(part 1 of 2)
# Autodesk Inventor assembly: ODrive S1 Housing Assembly
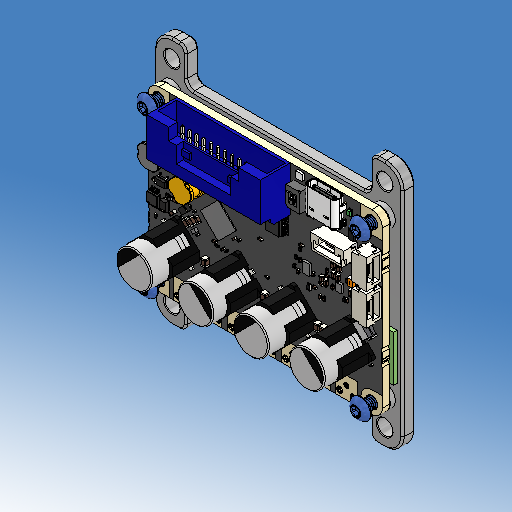
[picture p0: Inventor's stored thumbnail of the model, 512x512]
Saved by Autodesk Inventor 2025 (Build 290162000, 162)
## iProperties
Created: 2024-06-17
Part Number: ODrive S1 Housing Assembly
Description: STEP AP242
Document SubType Name: Assembly
Designer: seene
Title: 666fe0848788064f3eef2e7c
Preprocessor: ST-DEVELOPER v20
## Documents named in this file (550)
- C:\Users\seene\OneDrive\SBRT\Robocup Rescue\Chassis\Electronics Box\ODrive S1 Housing Assembly\ODrive S1 Housing Assembly.iam
- C:\Users\seene\OneDrive\SBRT\Robocup Rescue\Chassis\Electronics Box\ODrive S1 Housing Assembly\ODrive S1 Thermal Pad.ipt
- C:\Users\seene\OneDrive\SBRT\Robocup Rescue\Chassis\Electronics Box\ODrive S1 Housing Assembly\ODrive S1 Heatspreader.ipt
- C:\Users\seene\OneDrive\SBRT\Robocup Rescue\Chassis\Electronics Box\ODrive S1 Housing Assembly\90991A113_18-8 Stainless Steel Button Head Torx Screws.ipt
- C:\Users\seene\OneDrive\SBRT\Robocup Rescue\Chassis\Electronics Box\ODrive S1 Housing Assembly\ODrive S1 Cover.ipt
- C:\Users\seene\OneDrive\SBRT\Robocup Rescue\Chassis\Electronics Box\ODrive S1 Housing Assembly\C_0603_1608Metric_30.ipt
- C:\Users\seene\OneDrive\SBRT\Robocup Rescue\Chassis\Electronics Box\ODrive S1 Housing Assembly\C_0603_1608Metric_34.ipt
- C:\Users\seene\OneDrive\SBRT\Robocup Rescue\Chassis\Electronics Box\ODrive S1 Housing Assembly\C_0402_1005Metric_17.ipt
- C:\Users\seene\OneDrive\SBRT\Robocup Rescue\Chassis\Electronics Box\ODrive S1 Housing Assembly\C_0402_1005Metric_27.ipt
- C:\Users\seene\OneDrive\SBRT\Robocup Rescue\Chassis\Electronics Box\ODrive S1 Housing Assembly\C_0805_1MM_3.ipt
- C:\Users\seene\OneDrive\SBRT\Robocup Rescue\Chassis\Electronics Box\ODrive S1 Housing Assembly\_X2_8010632F54C130EA30FC30C97DDA03A6_X0_10_SIZE_CODE_G_4.ipt
- C:\Users\seene\OneDrive\SBRT\Robocup Rescue\Chassis\Electronics Box\ODrive S1 Housing Assembly\SOP_Advance(N)_(1)_7.ipt
- C:\Users\seene\OneDrive\SBRT\Robocup Rescue\Chassis\Electronics Box\ODrive S1 Housing Assembly\D_SOD-123F_3.ipt
- C:\Users\seene\OneDrive\SBRT\Robocup Rescue\Chassis\Electronics Box\ODrive S1 Housing Assembly\R_0402_1005Metric_63.ipt
- C:\Users\seene\OneDrive\SBRT\Robocup Rescue\Chassis\Electronics Box\ODrive S1 Housing Assembly\SOT23-3.ipt
- C:\Users\seene\OneDrive\SBRT\Robocup Rescue\Chassis\Electronics Box\ODrive S1 Housing Assembly\SOP_Advance(N)_(1)_2.ipt
- C:\Users\seene\OneDrive\SBRT\Robocup Rescue\Chassis\Electronics Box\ODrive S1 Housing Assembly\SOP_Advance(N)_(1)_5.ipt
- C:\Users\seene\OneDrive\SBRT\Robocup Rescue\Chassis\Electronics Box\ODrive S1 Housing Assembly\Open_CASCADE_STEP_translator_6.8_48.4.1_67.ipt
- C:\Users\seene\OneDrive\SBRT\Robocup Rescue\Chassis\Electronics Box\ODrive S1 Housing Assembly\R_0402_1005Metric_30.ipt
- C:\Users\seene\OneDrive\SBRT\Robocup Rescue\Chassis\Electronics Box\ODrive S1 Housing Assembly\R_0402_1005Metric_44.ipt
- C:\Users\seene\OneDrive\SBRT\Robocup Rescue\Chassis\Electronics Box\ODrive S1 Housing Assembly\R_0402_1005Metric_56.ipt
- C:\Users\seene\OneDrive\SBRT\Robocup Rescue\Chassis\Electronics Box\ODrive S1 Housing Assembly\Open_CASCADE_STEP_translator_6.8_48.4.1_3.ipt
- C:\Users\seene\OneDrive\SBRT\Robocup Rescue\Chassis\Electronics Box\ODrive S1 Housing Assembly\Open_CASCADE_STEP_translator_6.8_48.4.1_19.ipt
- C:\Users\seene\OneDrive\SBRT\Robocup Rescue\Chassis\Electronics Box\ODrive S1 Housing Assembly\Open_CASCADE_STEP_translator_6.8_48.4.1_35.ipt
- C:\Users\seene\OneDrive\SBRT\Robocup Rescue\Chassis\Electronics Box\ODrive S1 Housing Assembly\Open_CASCADE_STEP_translator_6.8_48.4.1_51.ipt
- C:\Users\seene\OneDrive\SBRT\Robocup Rescue\Chassis\Electronics Box\ODrive S1 Housing Assembly\LED_0603_APT1608_GREEN.ipt
- C:\Users\seene\OneDrive\SBRT\Robocup Rescue\Chassis\Electronics Box\ODrive S1 Housing Assembly\_X2_8010632F54C15EA7724803A6_X0_10_SIZE_CODE_G.ipt
- C:\Users\seene\OneDrive\SBRT\Robocup Rescue\Chassis\Electronics Box\ODrive S1 Housing Assembly\Open_CASCADE_STEP_translator_6.8_34.4.1_5.ipt
- C:\Users\seene\OneDrive\SBRT\Robocup Rescue\Chassis\Electronics Box\ODrive S1 Housing Assembly\Open_CASCADE_STEP_translator_6.8_41.4.1_2.ipt
- C:\Users\seene\OneDrive\SBRT\Robocup Rescue\Chassis\Electronics Box\ODrive S1 Housing Assembly\C_0402_1005Metric_8.ipt
- C:\Users\seene\OneDrive\SBRT\Robocup Rescue\Chassis\Electronics Box\ODrive S1 Housing Assembly\Cylinder_15.ipt
- C:\Users\seene\OneDrive\SBRT\Robocup Rescue\Chassis\Electronics Box\ODrive S1 Housing Assembly\SOT23-6.ipt
- C:\Users\seene\OneDrive\SBRT\Robocup Rescue\Chassis\Electronics Box\ODrive S1 Housing Assembly\C_0603_1608Metric_7.ipt
- C:\Users\seene\OneDrive\SBRT\Robocup Rescue\Chassis\Electronics Box\ODrive S1 Housing Assembly\Pins.ipt
- C:\Users\seene\OneDrive\SBRT\Robocup Rescue\Chassis\Electronics Box\ODrive S1 Housing Assembly\L_0603_1608Metric.ipt
- C:\Users\seene\OneDrive\SBRT\Robocup Rescue\Chassis\Electronics Box\ODrive S1 Housing Assembly\Open_CASCADE_STEP_translator_6.8_2.3.1_9.ipt
- C:\Users\seene\OneDrive\SBRT\Robocup Rescue\Chassis\Electronics Box\ODrive S1 Housing Assembly\Leader_2.ipt
- C:\Users\seene\OneDrive\SBRT\Robocup Rescue\Chassis\Electronics Box\ODrive S1 Housing Assembly\Open_CASCADE_STEP_translator_6.8_56.2.1.ipt
- C:\Users\seene\OneDrive\SBRT\Robocup Rescue\Chassis\Electronics Box\ODrive S1 Housing Assembly\Leader_4.ipt
- C:\Users\seene\OneDrive\SBRT\Robocup Rescue\Chassis\Electronics Box\ODrive S1 Housing Assembly\Leader_8.ipt
- C:\Users\seene\OneDrive\SBRT\Robocup Rescue\Chassis\Electronics Box\ODrive S1 Housing Assembly\C_0603_1608Metric_24.ipt
- C:\Users\seene\OneDrive\SBRT\Robocup Rescue\Chassis\Electronics Box\ODrive S1 Housing Assembly\D_SOD-123F.ipt
- C:\Users\seene\OneDrive\SBRT\Robocup Rescue\Chassis\Electronics Box\ODrive S1 Housing Assembly\_X2_8010632F54C15EA77248752888DC52A97AEF5B5003A6_X0_10_SIZE_CODE_G_3.ipt
- C:\Users\seene\OneDrive\SBRT\Robocup Rescue\Chassis\Electronics Box\ODrive S1 Housing Assembly\C_0603_1608Metric_13.ipt
- C:\Users\seene\OneDrive\SBRT\Robocup Rescue\Chassis\Electronics Box\ODrive S1 Housing Assembly\C_0603_1608Metric_26.ipt
- C:\Users\seene\OneDrive\SBRT\Robocup Rescue\Chassis\Electronics Box\ODrive S1 Housing Assembly\C_0603_1608Metric_15.ipt
- C:\Users\seene\OneDrive\SBRT\Robocup Rescue\Chassis\Electronics Box\ODrive S1 Housing Assembly\C_0805_2012Metric_6.ipt
- C:\Users\seene\OneDrive\SBRT\Robocup Rescue\Chassis\Electronics Box\ODrive S1 Housing Assembly\Extruded.ipt
- C:\Users\seene\OneDrive\SBRT\Robocup Rescue\Chassis\Electronics Box\ODrive S1 Housing Assembly\SOP_Advance(N)_(1)_6.ipt
- C:\Users\seene\OneDrive\SBRT\Robocup Rescue\Chassis\Electronics Box\ODrive S1 Housing Assembly\Open_CASCADE_STEP_translator_6.8_2.3.1_2.ipt
- C:\Users\seene\OneDrive\SBRT\Robocup Rescue\Chassis\Electronics Box\ODrive S1 Housing Assembly\C_0402_1005Metric_5.ipt
- C:\Users\seene\OneDrive\SBRT\Robocup Rescue\Chassis\Electronics Box\ODrive S1 Housing Assembly\C_0603_1608Metric_16.ipt
- C:\Users\seene\OneDrive\SBRT\Robocup Rescue\Chassis\Electronics Box\ODrive S1 Housing Assembly\Cylinder_9.ipt
- C:\Users\seene\OneDrive\SBRT\Robocup Rescue\Chassis\Electronics Box\ODrive S1 Housing Assembly\º¸½Å_2.ipt
- C:\Users\seene\OneDrive\SBRT\Robocup Rescue\Chassis\Electronics Box\ODrive S1 Housing Assembly\C_0402_1005Metric_21.ipt
- C:\Users\seene\OneDrive\SBRT\Robocup Rescue\Chassis\Electronics Box\ODrive S1 Housing Assembly\Cylinder_22.ipt
- C:\Users\seene\OneDrive\SBRT\Robocup Rescue\Chassis\Electronics Box\ODrive S1 Housing Assembly\Extruded_1.ipt
- C:\Users\seene\OneDrive\SBRT\Robocup Rescue\Chassis\Electronics Box\ODrive S1 Housing Assembly\SOP_Advance(N)_(1)_1.ipt
- C:\Users\seene\OneDrive\SBRT\Robocup Rescue\Chassis\Electronics Box\ODrive S1 Housing Assembly\SOP_Advance(N)_(1)_3.ipt
- C:\Users\seene\OneDrive\SBRT\Robocup Rescue\Chassis\Electronics Box\ODrive S1 Housing Assembly\R_0402_1005Metric_39.ipt
- C:\Users\seene\OneDrive\SBRT\Robocup Rescue\Chassis\Electronics Box\ODrive S1 Housing Assembly\R_0402_1005Metric_50.ipt
- C:\Users\seene\OneDrive\SBRT\Robocup Rescue\Chassis\Electronics Box\ODrive S1 Housing Assembly\HCS2512_L500_stp_3.ipt
- C:\Users\seene\OneDrive\SBRT\Robocup Rescue\Chassis\Electronics Box\ODrive S1 Housing Assembly\R_0402_1005Metric_68.ipt
- C:\Users\seene\OneDrive\SBRT\Robocup Rescue\Chassis\Electronics Box\ODrive S1 Housing Assembly\Open_CASCADE_STEP_translator_6.8_48.4.1_28.ipt
- C:\Users\seene\OneDrive\SBRT\Robocup Rescue\Chassis\Electronics Box\ODrive S1 Housing Assembly\Open_CASCADE_STEP_translator_6.8_48.4.1_44.ipt
- C:\Users\seene\OneDrive\SBRT\Robocup Rescue\Chassis\Electronics Box\ODrive S1 Housing Assembly\Open_CASCADE_STEP_translator_6.8_48.4.1_60.ipt
- C:\Users\seene\OneDrive\SBRT\Robocup Rescue\Chassis\Electronics Box\ODrive S1 Housing Assembly\R_0402_1005Metric_23.ipt
- C:\Users\seene\OneDrive\SBRT\Robocup Rescue\Chassis\Electronics Box\ODrive S1 Housing Assembly\Open_CASCADE_STEP_translator_6.8_56.4.1_7.ipt
- C:\Users\seene\OneDrive\SBRT\Robocup Rescue\Chassis\Electronics Box\ODrive S1 Housing Assembly\Leader_1.ipt
- C:\Users\seene\OneDrive\SBRT\Robocup Rescue\Chassis\Electronics Box\ODrive S1 Housing Assembly\Extruded_2.ipt
- C:\Users\seene\OneDrive\SBRT\Robocup Rescue\Chassis\Electronics Box\ODrive S1 Housing Assembly\Open_CASCADE_STEP_translator_6.8_48.4.1_12.ipt
- C:\Users\seene\OneDrive\SBRT\Robocup Rescue\Chassis\Electronics Box\ODrive S1 Housing Assembly\C_0402_1005Metric_36.ipt
- C:\Users\seene\OneDrive\SBRT\Robocup Rescue\Chassis\Electronics Box\ODrive S1 Housing Assembly\C_0402_1005Metric_43.ipt
- C:\Users\seene\OneDrive\SBRT\Robocup Rescue\Chassis\Electronics Box\ODrive S1 Housing Assembly\C_0402_1005Metric_16.ipt
- C:\Users\seene\OneDrive\SBRT\Robocup Rescue\Chassis\Electronics Box\ODrive S1 Housing Assembly\C_0402_1005Metric_26.ipt
- C:\Users\seene\OneDrive\SBRT\Robocup Rescue\Chassis\Electronics Box\ODrive S1 Housing Assembly\C_0805_1MM_3_1.ipt
- C:\Users\seene\OneDrive\SBRT\Robocup Rescue\Chassis\Electronics Box\ODrive S1 Housing Assembly\_X2_8010632F54C15EA77248752888DC52A97AEF5B5003A6_X0_10_SIZE_CODE_G_5.ipt
- C:\Users\seene\OneDrive\SBRT\Robocup Rescue\Chassis\Electronics Box\ODrive S1 Housing Assembly\SOP_Advance(N)_(1)_7_1.ipt
- C:\Users\seene\OneDrive\SBRT\Robocup Rescue\Chassis\Electronics Box\ODrive S1 Housing Assembly\L_0603_1608Metric_5.ipt
- C:\Users\seene\OneDrive\SBRT\Robocup Rescue\Chassis\Electronics Box\ODrive S1 Housing Assembly\R_0402_1005Metric_62.ipt
- C:\Users\seene\OneDrive\SBRT\Robocup Rescue\Chassis\Electronics Box\ODrive S1 Housing Assembly\R_0402_1005Metric_74.ipt
- C:\Users\seene\OneDrive\SBRT\Robocup Rescue\Chassis\Electronics Box\ODrive S1 Housing Assembly\SOP_Advance(N)_(1)_2_1.ipt
- C:\Users\seene\OneDrive\SBRT\Robocup Rescue\Chassis\Electronics Box\ODrive S1 Housing Assembly\SOP_Advance(N)_(1)_4.ipt
- C:\Users\seene\OneDrive\SBRT\Robocup Rescue\Chassis\Electronics Box\ODrive S1 Housing Assembly\Open_CASCADE_STEP_translator_6.8_48.4.1_66.ipt
- C:\Users\seene\OneDrive\SBRT\Robocup Rescue\Chassis\Electronics Box\ODrive S1 Housing Assembly\R_0402_1005Metric_29.ipt
- C:\Users\seene\OneDrive\SBRT\Robocup Rescue\Chassis\Electronics Box\ODrive S1 Housing Assembly\R_0603_1608Metric_1.ipt
- C:\Users\seene\OneDrive\SBRT\Robocup Rescue\Chassis\Electronics Box\ODrive S1 Housing Assembly\R_0402_1005Metric_55.ipt
- C:\Users\seene\OneDrive\SBRT\Robocup Rescue\Chassis\Electronics Box\ODrive S1 Housing Assembly\Open_CASCADE_STEP_translator_6.8_48.4.1_2.ipt
- C:\Users\seene\OneDrive\SBRT\Robocup Rescue\Chassis\Electronics Box\ODrive S1 Housing Assembly\Open_CASCADE_STEP_translator_6.8_48.4.1_18.ipt
- C:\Users\seene\OneDrive\SBRT\Robocup Rescue\Chassis\Electronics Box\ODrive S1 Housing Assembly\Open_CASCADE_STEP_translator_6.8_48.4.1_34.ipt
- C:\Users\seene\OneDrive\SBRT\Robocup Rescue\Chassis\Electronics Box\ODrive S1 Housing Assembly\Open_CASCADE_STEP_translator_6.8_48.4.1_50.ipt
- C:\Users\seene\OneDrive\SBRT\Robocup Rescue\Chassis\Electronics Box\ODrive S1 Housing Assembly\Leader_1_1.ipt
- C:\Users\seene\OneDrive\SBRT\Robocup Rescue\Chassis\Electronics Box\ODrive S1 Housing Assembly\Leader_3.ipt
- C:\Users\seene\OneDrive\SBRT\Robocup Rescue\Chassis\Electronics Box\ODrive S1 Housing Assembly\Leader_7.ipt
- C:\Users\seene\OneDrive\SBRT\Robocup Rescue\Chassis\Electronics Box\ODrive S1 Housing Assembly\B0-6.3-0-2512_2.ipt
- C:\Users\seene\OneDrive\SBRT\Robocup Rescue\Chassis\Electronics Box\ODrive S1 Housing Assembly\Cylinder_14.ipt
- C:\Users\seene\OneDrive\SBRT\Robocup Rescue\Chassis\Electronics Box\ODrive S1 Housing Assembly\Cylinder_8.ipt
- C:\Users\seene\OneDrive\SBRT\Robocup Rescue\Chassis\Electronics Box\ODrive S1 Housing Assembly\C_0603_1608Metric_6.ipt
- C:\Users\seene\OneDrive\SBRT\Robocup Rescue\Chassis\Electronics Box\ODrive S1 Housing Assembly\Pins_1.ipt
- C:\Users\seene\OneDrive\SBRT\Robocup Rescue\Chassis\Electronics Box\ODrive S1 Housing Assembly\R_0402_1005Metric_6.ipt
- C:\Users\seene\OneDrive\SBRT\Robocup Rescue\Chassis\Electronics Box\ODrive S1 Housing Assembly\Open_CASCADE_STEP_translator_6.8_2.3.1_8.ipt
- C:\Users\seene\OneDrive\SBRT\Robocup Rescue\Chassis\Electronics Box\ODrive S1 Housing Assembly\C_0805_1MM_2.ipt
- C:\Users\seene\OneDrive\SBRT\Robocup Rescue\Chassis\Electronics Box\ODrive S1 Housing Assembly\R_0402_1005Metric_10.ipt
- C:\Users\seene\OneDrive\SBRT\Robocup Rescue\Chassis\Electronics Box\ODrive S1 Housing Assembly\_X2_8010632F54C15EA77248752888DC52A97AEF5B5003A6_X0_10_SIZE_CODE_G_2.ipt
- C:\Users\seene\OneDrive\SBRT\Robocup Rescue\Chassis\Electronics Box\ODrive S1 Housing Assembly\C_0603_1608Metric_12.ipt
- C:\Users\seene\OneDrive\SBRT\Robocup Rescue\Chassis\Electronics Box\ODrive S1 Housing Assembly\C_0402_1005Metric_34.ipt
- C:\Users\seene\OneDrive\SBRT\Robocup Rescue\Chassis\Electronics Box\ODrive S1 Housing Assembly\R_0402_1005Metric_16.ipt
- C:\Users\seene\OneDrive\SBRT\Robocup Rescue\Chassis\Electronics Box\ODrive S1 Housing Assembly\C_0603_1608Metric_32.ipt
- C:\Users\seene\OneDrive\SBRT\Robocup Rescue\Chassis\Electronics Box\ODrive S1 Housing Assembly\Extruded_3.ipt
- C:\Users\seene\OneDrive\SBRT\Robocup Rescue\Chassis\Electronics Box\ODrive S1 Housing Assembly\SOP_Advance(N)_(1)_6_1.ipt
- C:\Users\seene\OneDrive\SBRT\Robocup Rescue\Chassis\Electronics Box\ODrive S1 Housing Assembly\Open_CASCADE_STEP_translator_6.8_2.3.1_1.ipt
- C:\Users\seene\OneDrive\SBRT\Robocup Rescue\Chassis\Electronics Box\ODrive S1 Housing Assembly\Open_CASCADE_STEP_translator_6.8_2.3.1_15.ipt
- C:\Users\seene\OneDrive\SBRT\Robocup Rescue\Chassis\Electronics Box\ODrive S1 Housing Assembly\C_0402_1005Metric_11.ipt
- C:\Users\seene\OneDrive\SBRT\Robocup Rescue\Chassis\Electronics Box\ODrive S1 Housing Assembly\Cylinder_8_1.ipt
- C:\Users\seene\OneDrive\SBRT\Robocup Rescue\Chassis\Electronics Box\ODrive S1 Housing Assembly\C_0402_1005Metric_20.ipt
- C:\Users\seene\OneDrive\SBRT\Robocup Rescue\Chassis\Electronics Box\ODrive S1 Housing Assembly\Cylinder_21.ipt
- C:\Users\seene\OneDrive\SBRT\Robocup Rescue\Chassis\Electronics Box\ODrive S1 Housing Assembly\Extruded_4.ipt
- C:\Users\seene\OneDrive\SBRT\Robocup Rescue\Chassis\Electronics Box\ODrive S1 Housing Assembly\SOP_Advance(N)_(1)_1_1.ipt
- C:\Users\seene\OneDrive\SBRT\Robocup Rescue\Chassis\Electronics Box\ODrive S1 Housing Assembly\SOP_Advance(N)_(1)_3_1.ipt
- C:\Users\seene\OneDrive\SBRT\Robocup Rescue\Chassis\Electronics Box\ODrive S1 Housing Assembly\R_0402_1005Metric_38.ipt
- C:\Users\seene\OneDrive\SBRT\Robocup Rescue\Chassis\Electronics Box\ODrive S1 Housing Assembly\R_0402_1005Metric_49.ipt
- C:\Users\seene\OneDrive\SBRT\Robocup Rescue\Chassis\Electronics Box\ODrive S1 Housing Assembly\HCS2512_L500_stp_3_1.ipt
- C:\Users\seene\OneDrive\SBRT\Robocup Rescue\Chassis\Electronics Box\ODrive S1 Housing Assembly\R_0402_1005Metric_67.ipt
- C:\Users\seene\OneDrive\SBRT\Robocup Rescue\Chassis\Electronics Box\ODrive S1 Housing Assembly\Open_CASCADE_STEP_translator_6.8_48.4.1_27.ipt
- C:\Users\seene\OneDrive\SBRT\Robocup Rescue\Chassis\Electronics Box\ODrive S1 Housing Assembly\Open_CASCADE_STEP_translator_6.8_48.4.1_43.ipt
- C:\Users\seene\OneDrive\SBRT\Robocup Rescue\Chassis\Electronics Box\ODrive S1 Housing Assembly\Open_CASCADE_STEP_translator_6.8_48.4.1_59.ipt
- C:\Users\seene\OneDrive\SBRT\Robocup Rescue\Chassis\Electronics Box\ODrive S1 Housing Assembly\R_0402_1005Metric_22.ipt
- C:\Users\seene\OneDrive\SBRT\Robocup Rescue\Chassis\Electronics Box\ODrive S1 Housing Assembly\Open_CASCADE_STEP_translator_6.8_56.4.1_6.ipt
- C:\Users\seene\OneDrive\SBRT\Robocup Rescue\Chassis\Electronics Box\ODrive S1 Housing Assembly\Leader.ipt
- C:\Users\seene\OneDrive\SBRT\Robocup Rescue\Chassis\Electronics Box\ODrive S1 Housing Assembly\Extruded_5.ipt
- C:\Users\seene\OneDrive\SBRT\Robocup Rescue\Chassis\Electronics Box\ODrive S1 Housing Assembly\Open_CASCADE_STEP_translator_6.8_48.4.1_11.ipt
- C:\Users\seene\OneDrive\SBRT\Robocup Rescue\Chassis\Electronics Box\ODrive S1 Housing Assembly\R_0402_1005Metric_12.ipt
- C:\Users\seene\OneDrive\SBRT\Robocup Rescue\Chassis\Electronics Box\ODrive S1 Housing Assembly\_X2_8010632F54C130B130FC30B903A6_X0_10x9.5L_SIDE_CODE_G.ipt
- C:\Users\seene\OneDrive\SBRT\Robocup Rescue\Chassis\Electronics Box\ODrive S1 Housing Assembly\Open_CASCADE_STEP_translator_6.8_34.4.1_4.ipt
- C:\Users\seene\OneDrive\SBRT\Robocup Rescue\Chassis\Electronics Box\ODrive S1 Housing Assembly\Open_CASCADE_STEP_translator_6.8_41.4.1_1.ipt
- C:\Users\seene\OneDrive\SBRT\Robocup Rescue\Chassis\Electronics Box\ODrive S1 Housing Assembly\C_0402_1005Metric_15.ipt
- C:\Users\seene\OneDrive\SBRT\Robocup Rescue\Chassis\Electronics Box\ODrive S1 Housing Assembly\C_0402_1005Metric_25.ipt
- C:\Users\seene\OneDrive\SBRT\Robocup Rescue\Chassis\Electronics Box\ODrive S1 Housing Assembly\C_0805_2012Metric_1.ipt
- C:\Users\seene\OneDrive\SBRT\Robocup Rescue\Chassis\Electronics Box\ODrive S1 Housing Assembly\_X2_8010632F54C15EA77248752888DC52A97AEF5B5003A6_X0_10_SIZE_CODE_G_4.ipt
- C:\Users\seene\OneDrive\SBRT\Robocup Rescue\Chassis\Electronics Box\ODrive S1 Housing Assembly\SOP_Advance(N)_(1)_7_2.ipt
- C:\Users\seene\OneDrive\SBRT\Robocup Rescue\Chassis\Electronics Box\ODrive S1 Housing Assembly\RES_0603_(1608_metric)_2.ipt
- C:\Users\seene\OneDrive\SBRT\Robocup Rescue\Chassis\Electronics Box\ODrive S1 Housing Assembly\R_0402_1005Metric_61.ipt
- C:\Users\seene\OneDrive\SBRT\Robocup Rescue\Chassis\Electronics Box\ODrive S1 Housing Assembly\R_0402_1005Metric_73.ipt
- C:\Users\seene\OneDrive\SBRT\Robocup Rescue\Chassis\Electronics Box\ODrive S1 Housing Assembly\SOP_Advance(N)_(1)_2_2.ipt
- C:\Users\seene\OneDrive\SBRT\Robocup Rescue\Chassis\Electronics Box\ODrive S1 Housing Assembly\SOP_Advance(N)_(1)_4_1.ipt
- C:\Users\seene\OneDrive\SBRT\Robocup Rescue\Chassis\Electronics Box\ODrive S1 Housing Assembly\Open_CASCADE_STEP_translator_6.8_48.4.1_65.ipt
- C:\Users\seene\OneDrive\SBRT\Robocup Rescue\Chassis\Electronics Box\ODrive S1 Housing Assembly\R_0402_1005Metric_28.ipt
- C:\Users\seene\OneDrive\SBRT\Robocup Rescue\Chassis\Electronics Box\ODrive S1 Housing Assembly\R_0603_1608Metric.ipt
- C:\Users\seene\OneDrive\SBRT\Robocup Rescue\Chassis\Electronics Box\ODrive S1 Housing Assembly\R_0402_1005Metric_54.ipt
- C:\Users\seene\OneDrive\SBRT\Robocup Rescue\Chassis\Electronics Box\ODrive S1 Housing Assembly\Open_CASCADE_STEP_translator_6.8_48.4.1_1.ipt
- C:\Users\seene\OneDrive\SBRT\Robocup Rescue\Chassis\Electronics Box\ODrive S1 Housing Assembly\Open_CASCADE_STEP_translator_6.8_48.4.1_17.ipt
- C:\Users\seene\OneDrive\SBRT\Robocup Rescue\Chassis\Electronics Box\ODrive S1 Housing Assembly\Open_CASCADE_STEP_translator_6.8_48.4.1_33.ipt
- C:\Users\seene\OneDrive\SBRT\Robocup Rescue\Chassis\Electronics Box\ODrive S1 Housing Assembly\Open_CASCADE_STEP_translator_6.8_48.4.1_49.ipt
- C:\Users\seene\OneDrive\SBRT\Robocup Rescue\Chassis\Electronics Box\ODrive S1 Housing Assembly\Leader_5.ipt
- C:\Users\seene\OneDrive\SBRT\Robocup Rescue\Chassis\Electronics Box\ODrive S1 Housing Assembly\Open_CASCADE_STEP_translator_6.8_41.4.1_7.ipt
- C:\Users\seene\OneDrive\SBRT\Robocup Rescue\Chassis\Electronics Box\ODrive S1 Housing Assembly\Leader_2_1.ipt
- C:\Users\seene\OneDrive\SBRT\Robocup Rescue\Chassis\Electronics Box\ODrive S1 Housing Assembly\Leader_6.ipt
- C:\Users\seene\OneDrive\SBRT\Robocup Rescue\Chassis\Electronics Box\ODrive S1 Housing Assembly\R_0402_1005Metric_9.ipt
- C:\Users\seene\OneDrive\SBRT\Robocup Rescue\Chassis\Electronics Box\ODrive S1 Housing Assembly\L_0603_1608Metric_3.ipt
- C:\Users\seene\OneDrive\SBRT\Robocup Rescue\Chassis\Electronics Box\ODrive S1 Housing Assembly\R_0402_1005Metric_15.ipt
- C:\Users\seene\OneDrive\SBRT\Robocup Rescue\Chassis\Electronics Box\ODrive S1 Housing Assembly\D_SOD-123F_2.ipt
- C:\Users\seene\OneDrive\SBRT\Robocup Rescue\Chassis\Electronics Box\ODrive S1 Housing Assembly\C_0402_1005Metric_35.ipt
- C:\Users\seene\OneDrive\SBRT\Robocup Rescue\Chassis\Electronics Box\ODrive S1 Housing Assembly\C_0402_1005Metric_42.ipt
- C:\Users\seene\OneDrive\SBRT\Robocup Rescue\Chassis\Electronics Box\ODrive S1 Housing Assembly\Cylinder_2.ipt
- C:\Users\seene\OneDrive\SBRT\Robocup Rescue\Chassis\Electronics Box\ODrive S1 Housing Assembly\Cylinder_1.ipt
- C:\Users\seene\OneDrive\SBRT\Robocup Rescue\Chassis\Electronics Box\ODrive S1 Housing Assembly\Cylinder.ipt
- C:\Users\seene\OneDrive\SBRT\Robocup Rescue\Chassis\Electronics Box\ODrive S1 Housing Assembly\C_0402_1005Metric_3.ipt
- C:\Users\seene\OneDrive\SBRT\Robocup Rescue\Chassis\Electronics Box\ODrive S1 Housing Assembly\C_0402_1005Metric_2.ipt
- C:\Users\seene\OneDrive\SBRT\Robocup Rescue\Chassis\Electronics Box\ODrive S1 Housing Assembly\C_0402_1005Metric_1.ipt
- C:\Users\seene\OneDrive\SBRT\Robocup Rescue\Chassis\Electronics Box\ODrive S1 Housing Assembly\C_0402_1005Metric.ipt
- C:\Users\seene\OneDrive\SBRT\Robocup Rescue\Chassis\Electronics Box\ODrive S1 Housing Assembly\Open_CASCADE_STEP_translator_6.8_2.3.1.ipt
- C:\Users\seene\OneDrive\SBRT\Robocup Rescue\Chassis\Electronics Box\ODrive S1 Housing Assembly\Open_CASCADE_STEP_translator_6.8_2.3.1_14.ipt
- C:\Users\seene\OneDrive\SBRT\Robocup Rescue\Chassis\Electronics Box\ODrive S1 Housing Assembly\Cylinder_7.ipt
- C:\Users\seene\OneDrive\SBRT\Robocup Rescue\Chassis\Electronics Box\ODrive S1 Housing Assembly\R_0402_1005Metric_4.ipt
- C:\Users\seene\OneDrive\SBRT\Robocup Rescue\Chassis\Electronics Box\ODrive S1 Housing Assembly\Cylinder_20.ipt
- C:\Users\seene\OneDrive\SBRT\Robocup Rescue\Chassis\Electronics Box\ODrive S1 Housing Assembly\R_0402_1005Metric_3.ipt
- C:\Users\seene\OneDrive\SBRT\Robocup Rescue\Chassis\Electronics Box\ODrive S1 Housing Assembly\Pins_2.ipt
- C:\Users\seene\OneDrive\SBRT\Robocup Rescue\Chassis\Electronics Box\ODrive S1 Housing Assembly\R_0402_1005Metric_2.ipt
- C:\Users\seene\OneDrive\SBRT\Robocup Rescue\Chassis\Electronics Box\ODrive S1 Housing Assembly\R_0402_1005Metric_1.ipt
- C:\Users\seene\OneDrive\SBRT\Robocup Rescue\Chassis\Electronics Box\ODrive S1 Housing Assembly\R_0402_1005Metric.ipt
- C:\Users\seene\OneDrive\SBRT\Robocup Rescue\Chassis\Electronics Box\ODrive S1 Housing Assembly\Open CASCADE STEP translator 6.8 1.1.1.1.ipt
- C:\Users\seene\OneDrive\SBRT\Robocup Rescue\Chassis\Electronics Box\ODrive S1 Housing Assembly\Pins_3.ipt
- C:\Users\seene\OneDrive\SBRT\Robocup Rescue\Chassis\Electronics Box\ODrive S1 Housing Assembly\Body.ipt
- C:\Users\seene\OneDrive\SBRT\Robocup Rescue\Chassis\Electronics Box\ODrive S1 Housing Assembly\Pins_4.ipt
- C:\Users\seene\OneDrive\SBRT\Robocup Rescue\Chassis\Electronics Box\ODrive S1 Housing Assembly\º¸½Å_6.ipt
- C:\Users\seene\OneDrive\SBRT\Robocup Rescue\Chassis\Electronics Box\ODrive S1 Housing Assembly\Ìú·½¿é_1.ipt
- C:\Users\seene\OneDrive\SBRT\Robocup Rescue\Chassis\Electronics Box\ODrive S1 Housing Assembly\Ìú·½¿é_2.ipt
- C:\Users\seene\OneDrive\SBRT\Robocup Rescue\Chassis\Electronics Box\ODrive S1 Housing Assembly\Ìú·½¿é_3.ipt
- C:\Users\seene\OneDrive\SBRT\Robocup Rescue\Chassis\Electronics Box\ODrive S1 Housing Assembly\Ìú·½¿é_4.ipt
- C:\Users\seene\OneDrive\SBRT\Robocup Rescue\Chassis\Electronics Box\ODrive S1 Housing Assembly\Ìú·½¿é_5.ipt
- C:\Users\seene\OneDrive\SBRT\Robocup Rescue\Chassis\Electronics Box\ODrive S1 Housing Assembly\Ìú·½¿é_6.ipt
- C:\Users\seene\OneDrive\SBRT\Robocup Rescue\Chassis\Electronics Box\ODrive S1 Housing Assembly\M3Ò»×ÖÆ½Ô²Í·ÂÝ¶¤_1.ipt
- C:\Users\seene\OneDrive\SBRT\Robocup Rescue\Chassis\Electronics Box\ODrive S1 Housing Assembly\M3Ò»×ÖÆ½Ô²Í·ÂÝ¶¤_2.ipt
- C:\Users\seene\OneDrive\SBRT\Robocup Rescue\Chassis\Electronics Box\ODrive S1 Housing Assembly\M3Ò»×ÖÆ½Ô²Í·ÂÝ¶¤_3.ipt
- C:\Users\seene\OneDrive\SBRT\Robocup Rescue\Chassis\Electronics Box\ODrive S1 Housing Assembly\M3Ò»×ÖÆ½Ô²Í·ÂÝ¶¤_4.ipt
- C:\Users\seene\OneDrive\SBRT\Robocup Rescue\Chassis\Electronics Box\ODrive S1 Housing Assembly\M3Ò»×ÖÆ½Ô²Í·ÂÝ¶¤_5.ipt
- C:\Users\seene\OneDrive\SBRT\Robocup Rescue\Chassis\Electronics Box\ODrive S1 Housing Assembly\M3Ò»×ÖÆ½Ô²Í·ÂÝ¶¤_6.ipt
- C:\Users\seene\OneDrive\SBRT\Robocup Rescue\Chassis\Electronics Box\ODrive S1 Housing Assembly\º¸½Å_4.ipt
- C:\Users\seene\OneDrive\SBRT\Robocup Rescue\Chassis\Electronics Box\ODrive S1 Housing Assembly\º¸½Å_5.ipt
- C:\Users\seene\OneDrive\SBRT\Robocup Rescue\Chassis\Electronics Box\ODrive S1 Housing Assembly\º¸½Å_3.ipt
- C:\Users\seene\OneDrive\SBRT\Robocup Rescue\Chassis\Electronics Box\ODrive S1 Housing Assembly\MX635-7.62-7P-ËÜ¼þ.ipt
- C:\Users\seene\OneDrive\SBRT\Robocup Rescue\Chassis\Electronics Box\ODrive S1 Housing Assembly\C_0402_1005Metric_38.ipt
- C:\Users\seene\OneDrive\SBRT\Robocup Rescue\Chassis\Electronics Box\ODrive S1 Housing Assembly\C_0603_1608Metric_20.ipt
- C:\Users\seene\OneDrive\SBRT\Robocup Rescue\Chassis\Electronics Box\ODrive S1 Housing Assembly\C_0402_1005Metric_30.ipt
- C:\Users\seene\OneDrive\SBRT\Robocup Rescue\Chassis\Electronics Box\ODrive S1 Housing Assembly\C_0805_1MM_4.ipt
- C:\Users\seene\OneDrive\SBRT\Robocup Rescue\Chassis\Electronics Box\ODrive S1 Housing Assembly\_X2_8010632F54C15EA77248752888DC52A97AEF5B5003A6_X0_10_SIZE_CODE_G_6.ipt
- C:\Users\seene\OneDrive\SBRT\Robocup Rescue\Chassis\Electronics Box\ODrive S1 Housing Assembly\srn6045.ipt
- C:\Users\seene\OneDrive\SBRT\Robocup Rescue\Chassis\Electronics Box\ODrive S1 Housing Assembly\D_SOD-123F_4.ipt
- C:\Users\seene\OneDrive\SBRT\Robocup Rescue\Chassis\Electronics Box\ODrive S1 Housing Assembly\SOP_Advance(N)_(1)_1_2.ipt
- C:\Users\seene\OneDrive\SBRT\Robocup Rescue\Chassis\Electronics Box\ODrive S1 Housing Assembly\SOP_Advance(N)_(1).ipt
- C:\Users\seene\OneDrive\SBRT\Robocup Rescue\Chassis\Electronics Box\ODrive S1 Housing Assembly\SOP_Advance(N)_(1)_4_2.ipt
- C:\Users\seene\OneDrive\SBRT\Robocup Rescue\Chassis\Electronics Box\ODrive S1 Housing Assembly\SOP_Advance(N)_(1)_3_2.ipt
- C:\Users\seene\OneDrive\SBRT\Robocup Rescue\Chassis\Electronics Box\ODrive S1 Housing Assembly\SOP_Advance(N)_(1)_6_2.ipt
- C:\Users\seene\OneDrive\SBRT\Robocup Rescue\Chassis\Electronics Box\ODrive S1 Housing Assembly\R_0402_1005Metric_43.ipt
- C:\Users\seene\OneDrive\SBRT\Robocup Rescue\Chassis\Electronics Box\ODrive S1 Housing Assembly\R_0402_1005Metric_36.ipt
- C:\Users\seene\OneDrive\SBRT\Robocup Rescue\Chassis\Electronics Box\ODrive S1 Housing Assembly\R_0402_1005Metric_53.ipt
- C:\Users\seene\OneDrive\SBRT\Robocup Rescue\Chassis\Electronics Box\ODrive S1 Housing Assembly\HCS2512_L500_stp.ipt
- C:\Users\seene\OneDrive\SBRT\Robocup Rescue\Chassis\Electronics Box\ODrive S1 Housing Assembly\R_0402_1005Metric_60.ipt
- C:\Users\seene\OneDrive\SBRT\Robocup Rescue\Chassis\Electronics Box\ODrive S1 Housing Assembly\HCS2512_L500_stp_2.ipt
- C:\Users\seene\OneDrive\SBRT\Robocup Rescue\Chassis\Electronics Box\ODrive S1 Housing Assembly\R_0402_1005Metric_72.ipt
- C:\Users\seene\OneDrive\SBRT\Robocup Rescue\Chassis\Electronics Box\ODrive S1 Housing Assembly\CRCW08057R50FKEAHP.ipt
- C:\Users\seene\OneDrive\SBRT\Robocup Rescue\Chassis\Electronics Box\ODrive S1 Housing Assembly\Open_CASCADE_STEP_translator_6.8_48.4.1_32.ipt
- C:\Users\seene\OneDrive\SBRT\Robocup Rescue\Chassis\Electronics Box\ODrive S1 Housing Assembly\Open_CASCADE_STEP_translator_6.8_48.4.1_25.ipt
- C:\Users\seene\OneDrive\SBRT\Robocup Rescue\Chassis\Electronics Box\ODrive S1 Housing Assembly\Open_CASCADE_STEP_translator_6.8_48.4.1_48.ipt
- C:\Users\seene\OneDrive\SBRT\Robocup Rescue\Chassis\Electronics Box\ODrive S1 Housing Assembly\Open_CASCADE_STEP_translator_6.8_48.4.1_41.ipt
- C:\Users\seene\OneDrive\SBRT\Robocup Rescue\Chassis\Electronics Box\ODrive S1 Housing Assembly\Open_CASCADE_STEP_translator_6.8_48.4.1_64.ipt
- C:\Users\seene\OneDrive\SBRT\Robocup Rescue\Chassis\Electronics Box\ODrive S1 Housing Assembly\Open_CASCADE_STEP_translator_6.8_48.4.1_57.ipt
- C:\Users\seene\OneDrive\SBRT\Robocup Rescue\Chassis\Electronics Box\ODrive S1 Housing Assembly\R_0402_1005Metric_27.ipt
- C:\Users\seene\OneDrive\SBRT\Robocup Rescue\Chassis\Electronics Box\ODrive S1 Housing Assembly\R_0402_1005Metric_20.ipt
- C:\Users\seene\OneDrive\SBRT\Robocup Rescue\Chassis\Electronics Box\ODrive S1 Housing Assembly\Leader_1_2.ipt
- C:\Users\seene\OneDrive\SBRT\Robocup Rescue\Chassis\Electronics Box\ODrive S1 Housing Assembly\Open_CASCADE_STEP_translator_6.8_56.4.1_4.ipt
- C:\Users\seene\OneDrive\SBRT\Robocup Rescue\Chassis\Electronics Box\ODrive S1 Housing Assembly\Leader_5_1.ipt
- C:\Users\seene\OneDrive\SBRT\Robocup Rescue\Chassis\Electronics Box\ODrive S1 Housing Assembly\Open_CASCADE_STEP_translator_6.8_48.4.1.ipt
- C:\Users\seene\OneDrive\SBRT\Robocup Rescue\Chassis\Electronics Box\ODrive S1 Housing Assembly\Leader_14.ipt
- C:\Users\seene\OneDrive\SBRT\Robocup Rescue\Chassis\Electronics Box\ODrive S1 Housing Assembly\Open_CASCADE_STEP_translator_6.8_48.4.1_16.ipt
- C:\Users\seene\OneDrive\SBRT\Robocup Rescue\Chassis\Electronics Box\ODrive S1 Housing Assembly\Open_CASCADE_STEP_translator_6.8_48.4.1_9.ipt
- C:\Users\seene\OneDrive\SBRT\Robocup Rescue\Chassis\Electronics Box\ODrive S1 Housing Assembly\C_0603_1608Metric_14.ipt
- C:\Users\seene\OneDrive\SBRT\Robocup Rescue\Chassis\Electronics Box\ODrive S1 Housing Assembly\SM04B-GHS-TB_1.ipt
- C:\Users\seene\OneDrive\SBRT\Robocup Rescue\Chassis\Electronics Box\ODrive S1 Housing Assembly\_X2_8010632F54C130EA30FC30C97DDA03A6_X0_10_SIZE_CODE_G_1.ipt
- C:\Users\seene\OneDrive\SBRT\Robocup Rescue\Chassis\Electronics Box\ODrive S1 Housing Assembly\R_0402_1005Metric_17.ipt
- C:\Users\seene\OneDrive\SBRT\Robocup Rescue\Chassis\Electronics Box\ODrive S1 Housing Assembly\Open_CASCADE_STEP_translator_6.8_35.1.1.ipt
- C:\Users\seene\OneDrive\SBRT\Robocup Rescue\Chassis\Electronics Box\ODrive S1 Housing Assembly\Open_CASCADE_STEP_translator_6.8_34.4.1_2.ipt
- C:\Users\seene\OneDrive\SBRT\Robocup Rescue\Chassis\Electronics Box\ODrive S1 Housing Assembly\Open_CASCADE_STEP_translator_6.8_41.4.1_6.ipt
- C:\Users\seene\OneDrive\SBRT\Robocup Rescue\Chassis\Electronics Box\ODrive S1 Housing Assembly\Thermal_Shape.ipt
- C:\Users\seene\OneDrive\SBRT\Robocup Rescue\Chassis\Electronics Box\ODrive S1 Housing Assembly\Cylinder_6.ipt
- C:\Users\seene\OneDrive\SBRT\Robocup Rescue\Chassis\Electronics Box\ODrive S1 Housing Assembly\B0-6.3-0-2512.ipt
- C:\Users\seene\OneDrive\SBRT\Robocup Rescue\Chassis\Electronics Box\ODrive S1 Housing Assembly\Cylinder_19.ipt
- C:\Users\seene\OneDrive\SBRT\Robocup Rescue\Chassis\Electronics Box\ODrive S1 Housing Assembly\Cylinder_2_1.ipt
- C:\Users\seene\OneDrive\SBRT\Robocup Rescue\Chassis\Electronics Box\ODrive S1 Housing Assembly\R_0402_1005Metric_8.ipt
- C:\Users\seene\OneDrive\SBRT\Robocup Rescue\Chassis\Electronics Box\ODrive S1 Housing Assembly\Cylinder_6_1.ipt
- C:\Users\seene\OneDrive\SBRT\Robocup Rescue\Chassis\Electronics Box\ODrive S1 Housing Assembly\C_0603_1608Metric_11.ipt
- C:\Users\seene\OneDrive\SBRT\Robocup Rescue\Chassis\Electronics Box\ODrive S1 Housing Assembly\C_0603_1608Metric_4.ipt
- C:\Users\seene\OneDrive\SBRT\Robocup Rescue\Chassis\Electronics Box\ODrive S1 Housing Assembly\Pins_5.ipt
- C:\Users\seene\OneDrive\SBRT\Robocup Rescue\Chassis\Electronics Box\ODrive S1 Housing Assembly\Open_CASCADE_STEP_translator_6.8_2.2.1.ipt
- C:\Users\seene\OneDrive\SBRT\Robocup Rescue\Chassis\Electronics Box\ODrive S1 Housing Assembly\lead_1.ipt
- C:\Users\seene\OneDrive\SBRT\Robocup Rescue\Chassis\Electronics Box\ODrive S1 Housing Assembly\Open_CASCADE_STEP_translator_6.8_2.3.1_13.ipt
- C:\Users\seene\OneDrive\SBRT\Robocup Rescue\Chassis\Electronics Box\ODrive S1 Housing Assembly\CRCW08057R50FKEAHP_1.ipt
- C:\Users\seene\OneDrive\SBRT\Robocup Rescue\Chassis\Electronics Box\ODrive S1 Housing Assembly\SOP_Advance(N)_(1)_8.ipt
- C:\Users\seene\OneDrive\SBRT\Robocup Rescue\Chassis\Electronics Box\ODrive S1 Housing Assembly\SOP_Advance(N)_(1)_3_3.ipt
- C:\Users\seene\OneDrive\SBRT\Robocup Rescue\Chassis\Electronics Box\ODrive S1 Housing Assembly\SOP_Advance(N)_(1)_5_1.ipt
- C:\Users\seene\OneDrive\SBRT\Robocup Rescue\Chassis\Electronics Box\ODrive S1 Housing Assembly\R_0402_1005Metric_18.ipt
- C:\Users\seene\OneDrive\SBRT\Robocup Rescue\Chassis\Electronics Box\ODrive S1 Housing Assembly\R_0402_1005Metric_34.ipt
- C:\Users\seene\OneDrive\SBRT\Robocup Rescue\Chassis\Electronics Box\ODrive S1 Housing Assembly\HCS2512_L500_stp_1.ipt
- C:\Users\seene\OneDrive\SBRT\Robocup Rescue\Chassis\Electronics Box\ODrive S1 Housing Assembly\HCS2512_L500_stp_2_1.ipt
- C:\Users\seene\OneDrive\SBRT\Robocup Rescue\Chassis\Electronics Box\ODrive S1 Housing Assembly\Open_CASCADE_STEP_translator_6.8_48.4.1_7.ipt
- C:\Users\seene\OneDrive\SBRT\Robocup Rescue\Chassis\Electronics Box\ODrive S1 Housing Assembly\Open_CASCADE_STEP_translator_6.8_48.4.1_23.ipt
- C:\Users\seene\OneDrive\SBRT\Robocup Rescue\Chassis\Electronics Box\ODrive S1 Housing Assembly\Open_CASCADE_STEP_translator_6.8_48.4.1_39.ipt
- C:\Users\seene\OneDrive\SBRT\Robocup Rescue\Chassis\Electronics Box\ODrive S1 Housing Assembly\Open_CASCADE_STEP_translator_6.8_48.4.1_55.ipt
- C:\Users\seene\OneDrive\SBRT\Robocup Rescue\Chassis\Electronics Box\ODrive S1 Housing Assembly\Open_CASCADE_STEP_translator_6.8_56.4.1_2.ipt
- C:\Users\seene\OneDrive\SBRT\Robocup Rescue\Chassis\Electronics Box\ODrive S1 Housing Assembly\Extruded_6.ipt
- C:\Users\seene\OneDrive\SBRT\Robocup Rescue\Chassis\Electronics Box\ODrive S1 Housing Assembly\Leader_12.ipt
- C:\Users\seene\OneDrive\SBRT\Robocup Rescue\Chassis\Electronics Box\ODrive S1 Housing Assembly\C_0402_1005Metric_33.ipt
- C:\Users\seene\OneDrive\SBRT\Robocup Rescue\Chassis\Electronics Box\ODrive S1 Housing Assembly\C_0805_1MM_1.ipt
- C:\Users\seene\OneDrive\SBRT\Robocup Rescue\Chassis\Electronics Box\ODrive S1 Housing Assembly\C_0603_1608Metric_2.ipt
- C:\Users\seene\OneDrive\SBRT\Robocup Rescue\Chassis\Electronics Box\ODrive S1 Housing Assembly\_X2_8010632F54C15EA7724803A6_X0_10_SIZE_CODE_G_2.ipt
- C:\Users\seene\OneDrive\SBRT\Robocup Rescue\Chassis\Electronics Box\ODrive S1 Housing Assembly\_X2_8010632F54C130B130FC30B903A6_X0_10x9.5L_SIDE_CODE_G_1.ipt
- C:\Users\seene\OneDrive\SBRT\Robocup Rescue\Chassis\Electronics Box\ODrive S1 Housing Assembly\SM04B-GHS-TB.ipt
- C:\Users\seene\OneDrive\SBRT\Robocup Rescue\Chassis\Electronics Box\ODrive S1 Housing Assembly\C_0805_2012Metric_5.ipt
- C:\Users\seene\OneDrive\SBRT\Robocup Rescue\Chassis\Electronics Box\ODrive S1 Housing Assembly\_X2_8010632F54C130EA30FC30C97DDA03A6_X0_10_SIZE_CODE_G_6.ipt
- C:\Users\seene\OneDrive\SBRT\Robocup Rescue\Chassis\Electronics Box\ODrive S1 Housing Assembly\B0-6.3-0-2512_5.ipt
- C:\Users\seene\OneDrive\SBRT\Robocup Rescue\Chassis\Electronics Box\ODrive S1 Housing Assembly\C_0805_2012Metric_8.ipt
- C:\Users\seene\OneDrive\SBRT\Robocup Rescue\Chassis\Electronics Box\ODrive S1 Housing Assembly\C_0402_1005Metric_40.ipt
- C:\Users\seene\OneDrive\SBRT\Robocup Rescue\Chassis\Electronics Box\ODrive S1 Housing Assembly\Open_CASCADE_STEP_translator_6.8_34.4.1.ipt
- C:\Users\seene\OneDrive\SBRT\Robocup Rescue\Chassis\Electronics Box\ODrive S1 Housing Assembly\SOP_Advance(N)_(1)_7_3.ipt
- C:\Users\seene\OneDrive\SBRT\Robocup Rescue\Chassis\Electronics Box\ODrive S1 Housing Assembly\Open_CASCADE_STEP_translator_6.8_2.3.1_6.ipt
- C:\Users\seene\OneDrive\SBRT\Robocup Rescue\Chassis\Electronics Box\ODrive S1 Housing Assembly\RES_0603_(1608_metric)_1.ipt
- C:\Users\seene\OneDrive\SBRT\Robocup Rescue\Chassis\Electronics Box\ODrive S1 Housing Assembly\S30B-PUDSS-1.ipt
- C:\Users\seene\OneDrive\SBRT\Robocup Rescue\Chassis\Electronics Box\ODrive S1 Housing Assembly\L_0603_1608Metric_1.ipt
- C:\Users\seene\OneDrive\SBRT\Robocup Rescue\Chassis\Electronics Box\ODrive S1 Housing Assembly\C_0603_1608Metric_17.ipt
- C:\Users\seene\OneDrive\SBRT\Robocup Rescue\Chassis\Electronics Box\ODrive S1 Housing Assembly\Extruded_7.ipt
- C:\Users\seene\OneDrive\SBRT\Robocup Rescue\Chassis\Electronics Box\ODrive S1 Housing Assembly\Cylinder_3.ipt
- C:\Users\seene\OneDrive\SBRT\Robocup Rescue\Chassis\Electronics Box\ODrive S1 Housing Assembly\º¸½Å.ipt
- C:\Users\seene\OneDrive\SBRT\Robocup Rescue\Chassis\Electronics Box\ODrive S1 Housing Assembly\C_0402_1005Metric_24.ipt
- C:\Users\seene\OneDrive\SBRT\Robocup Rescue\Chassis\Electronics Box\ODrive S1 Housing Assembly\C_0603_1608Metric_22.ipt
- C:\Users\seene\OneDrive\SBRT\Robocup Rescue\Chassis\Electronics Box\ODrive S1 Housing Assembly\Cylinder_4.ipt
- C:\Users\seene\OneDrive\SBRT\Robocup Rescue\Chassis\Electronics Box\ODrive S1 Housing Assembly\Open_CASCADE_STEP_translator_6.8_13.2.1.ipt
- C:\Users\seene\OneDrive\SBRT\Robocup Rescue\Chassis\Electronics Box\ODrive S1 Housing Assembly\C_0402_1005Metric_37.ipt
- C:\Users\seene\OneDrive\SBRT\Robocup Rescue\Chassis\Electronics Box\ODrive S1 Housing Assembly\C_0402_1005Metric_18.ipt
- C:\Users\seene\OneDrive\SBRT\Robocup Rescue\Chassis\Electronics Box\ODrive S1 Housing Assembly\C_0402_1005Metric_29.ipt
- C:\Users\seene\OneDrive\SBRT\Robocup Rescue\Chassis\Electronics Box\ODrive S1 Housing Assembly\C_0805_1MM_4_1.ipt
- C:\Users\seene\OneDrive\SBRT\Robocup Rescue\Chassis\Electronics Box\ODrive S1 Housing Assembly\_X2_8010632F54C15EA7724803A6_X0_10_SIZE_CODE_G_3.ipt
- C:\Users\seene\OneDrive\SBRT\Robocup Rescue\Chassis\Electronics Box\ODrive S1 Housing Assembly\ASMPH-0806_1.ipt
- C:\Users\seene\OneDrive\SBRT\Robocup Rescue\Chassis\Electronics Box\ODrive S1 Housing Assembly\SW3dPS-DO-214AC_SMA.ipt
- C:\Users\seene\OneDrive\SBRT\Robocup Rescue\Chassis\Electronics Box\ODrive S1 Housing Assembly\R_0402_1005Metric_42.ipt
- C:\Users\seene\OneDrive\SBRT\Robocup Rescue\Chassis\Electronics Box\ODrive S1 Housing Assembly\R_0402_1005Metric_35.ipt
- C:\Users\seene\OneDrive\SBRT\Robocup Rescue\Chassis\Electronics Box\ODrive S1 Housing Assembly\R_0402_1005Metric_52.ipt
- C:\Users\seene\OneDrive\SBRT\Robocup Rescue\Chassis\Electronics Box\ODrive S1 Housing Assembly\HCS2512_L500_stp_4.ipt
- C:\Users\seene\OneDrive\SBRT\Robocup Rescue\Chassis\Electronics Box\ODrive S1 Housing Assembly\R_0402_1005Metric_59.ipt
- C:\Users\seene\OneDrive\SBRT\Robocup Rescue\Chassis\Electronics Box\ODrive S1 Housing Assembly\HCS2512_L500_stp_2_2.ipt
- C:\Users\seene\OneDrive\SBRT\Robocup Rescue\Chassis\Electronics Box\ODrive S1 Housing Assembly\R_0402_1005Metric_71.ipt
- C:\Users\seene\OneDrive\SBRT\Robocup Rescue\Chassis\Electronics Box\ODrive S1 Housing Assembly\CRCW08057R50FKEAHP_2.ipt
- C:\Users\seene\OneDrive\SBRT\Robocup Rescue\Chassis\Electronics Box\ODrive S1 Housing Assembly\Open_CASCADE_STEP_translator_6.8_48.4.1_31.ipt
- C:\Users\seene\OneDrive\SBRT\Robocup Rescue\Chassis\Electronics Box\ODrive S1 Housing Assembly\Open_CASCADE_STEP_translator_6.8_48.4.1_24.ipt
- C:\Users\seene\OneDrive\SBRT\Robocup Rescue\Chassis\Electronics Box\ODrive S1 Housing Assembly\Open_CASCADE_STEP_translator_6.8_48.4.1_47.ipt
- C:\Users\seene\OneDrive\SBRT\Robocup Rescue\Chassis\Electronics Box\ODrive S1 Housing Assembly\Open_CASCADE_STEP_translator_6.8_48.4.1_40.ipt
- C:\Users\seene\OneDrive\SBRT\Robocup Rescue\Chassis\Electronics Box\ODrive S1 Housing Assembly\Open_CASCADE_STEP_translator_6.8_48.4.1_63.ipt
- C:\Users\seene\OneDrive\SBRT\Robocup Rescue\Chassis\Electronics Box\ODrive S1 Housing Assembly\Open_CASCADE_STEP_translator_6.8_48.4.1_56.ipt
- C:\Users\seene\OneDrive\SBRT\Robocup Rescue\Chassis\Electronics Box\ODrive S1 Housing Assembly\R_0402_1005Metric_26.ipt
- C:\Users\seene\OneDrive\SBRT\Robocup Rescue\Chassis\Electronics Box\ODrive S1 Housing Assembly\R_0402_1005Metric_19.ipt
- C:\Users\seene\OneDrive\SBRT\Robocup Rescue\Chassis\Electronics Box\ODrive S1 Housing Assembly\Leader_9.ipt
- C:\Users\seene\OneDrive\SBRT\Robocup Rescue\Chassis\Electronics Box\ODrive S1 Housing Assembly\Open_CASCADE_STEP_translator_6.8_56.4.1_3.ipt
- C:\Users\seene\OneDrive\SBRT\Robocup Rescue\Chassis\Electronics Box\ODrive S1 Housing Assembly\Leader_4_1.ipt
- C:\Users\seene\OneDrive\SBRT\Robocup Rescue\Chassis\Electronics Box\ODrive S1 Housing Assembly\Extruded_8.ipt
- C:\Users\seene\OneDrive\SBRT\Robocup Rescue\Chassis\Electronics Box\ODrive S1 Housing Assembly\Thermal_Shape_1.ipt
- C:\Users\seene\OneDrive\SBRT\Robocup Rescue\Chassis\Electronics Box\ODrive S1 Housing Assembly\Leader_13.ipt
- C:\Users\seene\OneDrive\SBRT\Robocup Rescue\Chassis\Electronics Box\ODrive S1 Housing Assembly\Open_CASCADE_STEP_translator_6.8_48.4.1_15.ipt
- C:\Users\seene\OneDrive\SBRT\Robocup Rescue\Chassis\Electronics Box\ODrive S1 Housing Assembly\Open_CASCADE_STEP_translator_6.8_48.4.1_8.ipt
- C:\Users\seene\OneDrive\SBRT\Robocup Rescue\Chassis\Electronics Box\ODrive S1 Housing Assembly\R_0402_1005Metric_14.ipt
- C:\Users\seene\OneDrive\SBRT\Robocup Rescue\Chassis\Electronics Box\ODrive S1 Housing Assembly\_X2_8010632F54C130EA30FC30C97DDA03A6_X0_10_SIZE_CODE_G.ipt
- C:\Users\seene\OneDrive\SBRT\Robocup Rescue\Chassis\Electronics Box\ODrive S1 Housing Assembly\B0-6.3-0-2512_6.ipt
- C:\Users\seene\OneDrive\SBRT\Robocup Rescue\Chassis\Electronics Box\ODrive S1 Housing Assembly\SOT23-5.ipt
- C:\Users\seene\OneDrive\SBRT\Robocup Rescue\Chassis\Electronics Box\ODrive S1 Housing Assembly\Open_CASCADE_STEP_translator_6.8_34.4.1_1.ipt
- C:\Users\seene\OneDrive\SBRT\Robocup Rescue\Chassis\Electronics Box\ODrive S1 Housing Assembly\Open_CASCADE_STEP_translator_6.8_41.4.1_5.ipt
- C:\Users\seene\OneDrive\SBRT\Robocup Rescue\Chassis\Electronics Box\ODrive S1 Housing Assembly\Open_CASCADE_STEP_translator_6.8_41.2.1.ipt
- C:\Users\seene\OneDrive\SBRT\Robocup Rescue\Chassis\Electronics Box\ODrive S1 Housing Assembly\Cylinder_5.ipt
- C:\Users\seene\OneDrive\SBRT\Robocup Rescue\Chassis\Electronics Box\ODrive S1 Housing Assembly\L_0603_1608Metric_2.ipt
- C:\Users\seene\OneDrive\SBRT\Robocup Rescue\Chassis\Electronics Box\ODrive S1 Housing Assembly\Cylinder_18.ipt
- C:\Users\seene\OneDrive\SBRT\Robocup Rescue\Chassis\Electronics Box\ODrive S1 Housing Assembly\Cylinder_1_1.ipt
- C:\Users\seene\OneDrive\SBRT\Robocup Rescue\Chassis\Electronics Box\ODrive S1 Housing Assembly\Open_CASCADE_STEP_translator_6.8_10.2.1.ipt
- C:\Users\seene\OneDrive\SBRT\Robocup Rescue\Chassis\Electronics Box\ODrive S1 Housing Assembly\Cylinder_5_1.ipt
- C:\Users\seene\OneDrive\SBRT\Robocup Rescue\Chassis\Electronics Box\ODrive S1 Housing Assembly\C_0603_1608Metric_10.ipt
- C:\Users\seene\OneDrive\SBRT\Robocup Rescue\Chassis\Electronics Box\ODrive S1 Housing Assembly\C_0603_1608Metric_3.ipt
- C:\Users\seene\OneDrive\SBRT\Robocup Rescue\Chassis\Electronics Box\ODrive S1 Housing Assembly\Pins_6.ipt
- C:\Users\seene\OneDrive\SBRT\Robocup Rescue\Chassis\Electronics Box\ODrive S1 Housing Assembly\lead.ipt
- C:\Users\seene\OneDrive\SBRT\Robocup Rescue\Chassis\Electronics Box\ODrive S1 Housing Assembly\Open_CASCADE_STEP_translator_6.8_2.3.1_12.ipt
- C:\Users\seene\OneDrive\SBRT\Robocup Rescue\Chassis\Electronics Box\ODrive S1 Housing Assembly\Open_CASCADE_STEP_translator_6.8_2.3.1_7.ipt
- C:\Users\seene\OneDrive\SBRT\Robocup Rescue\Chassis\Electronics Box\ODrive S1 Housing Assembly\CRCW08057R50FKEAHP_3.ipt
- C:\Users\seene\OneDrive\SBRT\Robocup Rescue\Chassis\Electronics Box\ODrive S1 Housing Assembly\SOP_Advance(N)_(1)_9.ipt
- C:\Users\seene\OneDrive\SBRT\Robocup Rescue\Chassis\Electronics Box\ODrive S1 Housing Assembly\SOP_Advance(N)_(1)_2_3.ipt
- C:\Users\seene\OneDrive\SBRT\Robocup Rescue\Chassis\Electronics Box\ODrive S1 Housing Assembly\SOP_Advance(N)_(1)_5_2.ipt
- C:\Users\seene\OneDrive\SBRT\Robocup Rescue\Chassis\Electronics Box\ODrive S1 Housing Assembly\_Dual_s_1.ipt
- C:\Users\seene\OneDrive\SBRT\Robocup Rescue\Chassis\Electronics Box\ODrive S1 Housing Assembly\R_0402_1005Metric_33.ipt
- C:\Users\seene\OneDrive\SBRT\Robocup Rescue\Chassis\Electronics Box\ODrive S1 Housing Assembly\R_0402_1005Metric_47.ipt
- C:\Users\seene\OneDrive\SBRT\Robocup Rescue\Chassis\Electronics Box\ODrive S1 Housing Assembly\HCS2512_L500_stp_1_1.ipt
- C:\Users\seene\OneDrive\SBRT\Robocup Rescue\Chassis\Electronics Box\ODrive S1 Housing Assembly\Open_CASCADE_STEP_translator_6.8_48.4.1_6.ipt
- C:\Users\seene\OneDrive\SBRT\Robocup Rescue\Chassis\Electronics Box\ODrive S1 Housing Assembly\Open_CASCADE_STEP_translator_6.8_48.4.1_22.ipt
- C:\Users\seene\OneDrive\SBRT\Robocup Rescue\Chassis\Electronics Box\ODrive S1 Housing Assembly\Open_CASCADE_STEP_translator_6.8_48.4.1_38.ipt
- C:\Users\seene\OneDrive\SBRT\Robocup Rescue\Chassis\Electronics Box\ODrive S1 Housing Assembly\Open_CASCADE_STEP_translator_6.8_48.4.1_54.ipt
- C:\Users\seene\OneDrive\SBRT\Robocup Rescue\Chassis\Electronics Box\ODrive S1 Housing Assembly\Leader_5_2.ipt
- C:\Users\seene\OneDrive\SBRT\Robocup Rescue\Chassis\Electronics Box\ODrive S1 Housing Assembly\Open_CASCADE_STEP_translator_6.8_56.4.1_1.ipt
- C:\Users\seene\OneDrive\SBRT\Robocup Rescue\Chassis\Electronics Box\ODrive S1 Housing Assembly\Leader_7_1.ipt
- C:\Users\seene\OneDrive\SBRT\Robocup Rescue\Chassis\Electronics Box\ODrive S1 Housing Assembly\Leader_11.ipt
- C:\Users\seene\OneDrive\SBRT\Robocup Rescue\Chassis\Electronics Box\ODrive S1 Housing Assembly\C_0402_1005Metric_32.ipt
- C:\Users\seene\OneDrive\SBRT\Robocup Rescue\Chassis\Electronics Box\ODrive S1 Housing Assembly\C_0805_1MM_1_1.ipt
- C:\Users\seene\OneDrive\SBRT\Robocup Rescue\Chassis\Electronics Box\ODrive S1 Housing Assembly\Extruded_9.ipt
- C:\Users\seene\OneDrive\SBRT\Robocup Rescue\Chassis\Electronics Box\ODrive S1 Housing Assembly\_X2_8010632F54C130B130FC30B903A6_X0_10x9.5L_SIDE_CODE_G_2.ipt
- C:\Users\seene\OneDrive\SBRT\Robocup Rescue\Chassis\Electronics Box\ODrive S1 Housing Assembly\C_0805_2012Metric_4.ipt
- C:\Users\seene\OneDrive\SBRT\Robocup Rescue\Chassis\Electronics Box\ODrive S1 Housing Assembly\D_SOD-123F_1.ipt
- C:\Users\seene\OneDrive\SBRT\Robocup Rescue\Chassis\Electronics Box\ODrive S1 Housing Assembly\C_0603_1608Metric_29.ipt
- C:\Users\seene\OneDrive\SBRT\Robocup Rescue\Chassis\Electronics Box\ODrive S1 Housing Assembly\_X2_8010632F54C15EA77248752888DC52A97AEF5B5003A6_X0_10_SIZE_CODE_G_7.ipt
- C:\Users\seene\OneDrive\SBRT\Robocup Rescue\Chassis\Electronics Box\ODrive S1 Housing Assembly\B0-6.3-0-2512_4.ipt
- C:\Users\seene\OneDrive\SBRT\Robocup Rescue\Chassis\Electronics Box\ODrive S1 Housing Assembly\C_0805_2012Metric_7.ipt
- C:\Users\seene\OneDrive\SBRT\Robocup Rescue\Chassis\Electronics Box\ODrive S1 Housing Assembly\C_0402_1005Metric_39.ipt
- C:\Users\seene\OneDrive\SBRT\Robocup Rescue\Chassis\Electronics Box\ODrive S1 Housing Assembly\Thermal_Shape_2.ipt
- C:\Users\seene\OneDrive\SBRT\Robocup Rescue\Chassis\Electronics Box\ODrive S1 Housing Assembly\SOP_Advance(N)_(1)_7_4.ipt
- C:\Users\seene\OneDrive\SBRT\Robocup Rescue\Chassis\Electronics Box\ODrive S1 Housing Assembly\Open_CASCADE_STEP_translator_6.8_2.3.1_5.ipt
- C:\Users\seene\OneDrive\SBRT\Robocup Rescue\Chassis\Electronics Box\ODrive S1 Housing Assembly\L_0603_1608Metric_4.ipt
- C:\Users\seene\OneDrive\SBRT\Robocup Rescue\Chassis\Electronics Box\ODrive S1 Housing Assembly\srn6045_1.ipt
- C:\Users\seene\OneDrive\SBRT\Robocup Rescue\Chassis\Electronics Box\ODrive S1 Housing Assembly\C_0402_1005Metric_7.ipt
- C:\Users\seene\OneDrive\SBRT\Robocup Rescue\Chassis\Electronics Box\ODrive S1 Housing Assembly\C_0402_1005Metric_14.ipt
- C:\Users\seene\OneDrive\SBRT\Robocup Rescue\Chassis\Electronics Box\ODrive S1 Housing Assembly\Extruded_10.ipt
- C:\Users\seene\OneDrive\SBRT\Robocup Rescue\Chassis\Electronics Box\ODrive S1 Housing Assembly\Cylinder_12.ipt
- C:\Users\seene\OneDrive\SBRT\Robocup Rescue\Chassis\Electronics Box\ODrive S1 Housing Assembly\Ìú·½¿é.ipt
- C:\Users\seene\OneDrive\SBRT\Robocup Rescue\Chassis\Electronics Box\ODrive S1 Housing Assembly\C_0603_1608Metric_23.ipt
- C:\Users\seene\OneDrive\SBRT\Robocup Rescue\Chassis\Electronics Box\ODrive S1 Housing Assembly\C_0603_1608Metric_21.ipt
- C:\Users\seene\OneDrive\SBRT\Robocup Rescue\Chassis\Electronics Box\ODrive S1 Housing Assembly\Cylinder_3_1.ipt
- C:\Users\seene\OneDrive\SBRT\Robocup Rescue\Chassis\Electronics Box\ODrive S1 Housing Assembly\SOP_Advance(N)_(1)_1_3.ipt
- C:\Users\seene\OneDrive\SBRT\Robocup Rescue\Chassis\Electronics Box\ODrive S1 Housing Assembly\SOP_Advance(N)_(1)_10.ipt
- C:\Users\seene\OneDrive\SBRT\Robocup Rescue\Chassis\Electronics Box\ODrive S1 Housing Assembly\SOP_Advance(N)_(1)_4_3.ipt
- C:\Users\seene\OneDrive\SBRT\Robocup Rescue\Chassis\Electronics Box\ODrive S1 Housing Assembly\SOP_Advance(N)_(1)_3_4.ipt
- C:\Users\seene\OneDrive\SBRT\Robocup Rescue\Chassis\Electronics Box\ODrive S1 Housing Assembly\SOP_Advance(N)_(1)_5_3.ipt
- C:\Users\seene\OneDrive\SBRT\Robocup Rescue\Chassis\Electronics Box\ODrive S1 Housing Assembly\C_0805_1MM_5.ipt
- C:\Users\seene\OneDrive\SBRT\Robocup Rescue\Chassis\Electronics Box\ODrive S1 Housing Assembly\C_0603_1608Metric_19.ipt
- C:\Users\seene\OneDrive\SBRT\Robocup Rescue\Chassis\Electronics Box\ODrive S1 Housing Assembly\C_0402_1005Metric_28.ipt